# Autodesk Inventor assembly: JigAssembly
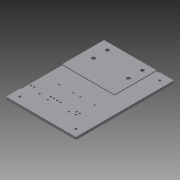
[picture p0: Inventor's stored thumbnail of the model, 180x180]
Saved by Autodesk Inventor 2014 (Build 180170000, 170)
## iProperties
Created: 2014-10-04
Part Number: JigAssembly
Document SubType Name: Assembly
Designer: Rachel
Author: Rachel
## Documents named in this file (4)
- C:\Users\Rachel\Desktop\GitHub\reflow-structure\reflow_jig\JigAssembly.iam
- C:\Users\Rachel\Desktop\GitHub\reflow-structure\reflow_jig\bottomLayer.ipt
- C:\Users\Rachel\Desktop\GitHub\reflow-structure\reflow_jig\topLayer.ipt
- C:\Users\Rachel\Desktop\GitHub\reflow-structure\reflow_jig\slider.ipt
## Components (3 placed, 3 different names)
1. bottomLayer:1 — Mate:1, Mate:2, Flush:1, Mate:3, Mate:4
2. topLayer:1 — Mate:1, Mate:2, Flush:1
3. slider:1 — Mate:3, Mate:4
## Relationships (5: Mate 4, Flush 1)
- Mate:1: bottomLayer:1 ↔ topLayer:1
- Mate:2: bottomLayer:1 ↔ topLayer:1
- Flush:1: bottomLayer:1 ↔ topLayer:1
- Mate:3: bottomLayer:1 ↔ slider:1
- Mate:4: bottomLayer:1 ↔ slider:1
